# Autodesk Inventor assembly: GFRP_T2_03
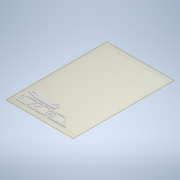
[picture p0: Inventor's stored thumbnail of the model, 180x180]
Saved by Autodesk Inventor 2020 (Build 240168000, 168)
## iProperties
Created: 2021-08-27
Part Number: GFRP_T2_03
Document SubType Name: Assembly
Designer: Masato
Author: Masato
## Documents named in this file (4)
- C:\Users\naoki\Documents\Inventor\CitBrains\git_clone\OpenPlatform4_0\CAM\OpenPlatform_ver3_0\cam\GFRP_T2_03.iam
- C:\Users\naoki\Documents\Inventor\CitBrains\git_clone\OpenPlatform4_0\ver4_0_cam_branch\OpenPlatform_ver3_0\cam\Disposable_Board.ipt
- C:\Users\naoki\Documents\Inventor\CitBrains\git_clone\OpenPlatform4_0\ver4_0_cam_branch\OpenPlatform_ver3_0\UpperBody\Arm\UpperArm_side_frame.ipt
- C:\Users\naoki\Documents\Inventor\CitBrains\git_clone\OpenPlatform4_0\ver4_0_cam_branch\OpenPlatform_ver3_0\UpperBody\Arm\ForeArm_inside_frame.ipt
## Components (5 placed, 3 different names)
1. Disposable_Board:1 — メイト:2, メイト:1, フラッシュ:1, フラッシュ:2, フラッシュ:3, フラッシュ:4
2. ForeArm_inside_frame:1 — メイト:4, フラッシュ:6, メイト:7
3. UpperArm_side_frame:2 — メイト:6, フラッシュ:5, 正接:1, メイト:9, フラッシュ:7
4. UpperArm_side_frame:1 — メイト:5, フラッシュ:3, フラッシュ:4, 正接:1, フラッシュ:5, フラッシュ:6, メイト:7
5. UpperArm_side_frame:3 — メイト:8, メイト:9, フラッシュ:7
## Relationships (16: Mate 8, Flush 7, Tangent 1)
- メイト:2 [Mate]: Disposable_Board:1
- メイト:1 [Mate]: Disposable_Board:1
- フラッシュ:1 [Flush]: Disposable_Board:1
- フラッシュ:2 [Flush]: Disposable_Board:1
- メイト:4 [Mate]: ForeArm_inside_frame:1
- メイト:5 [Mate]: UpperArm_side_frame:1
- フラッシュ:3 [Flush] (2 mm): Disposable_Board:1 ↔ UpperArm_side_frame:1
- フラッシュ:4 [Flush] (2 mm): Disposable_Board:1 ↔ UpperArm_side_frame:1
- メイト:6 [Mate]: UpperArm_side_frame:2
- フラッシュ:5 [Flush]: UpperArm_side_frame:2 ↔ UpperArm_side_frame:1
- 正接:1 [Tangent] (2.5 mm): UpperArm_side_frame:2 ↔ UpperArm_side_frame:1
- フラッシュ:6 [Flush]: ForeArm_inside_frame:1 ↔ UpperArm_side_frame:1
- メイト:7 [Mate] (2.5 mm): ForeArm_inside_frame:1 ↔ UpperArm_side_frame:1
- メイト:8 [Mate]: UpperArm_side_frame:3
- メイト:9 [Mate] (2.5 mm): UpperArm_side_frame:2 ↔ UpperArm_side_frame:3
- フラッシュ:7 [Flush]: UpperArm_side_frame:2 ↔ UpperArm_side_frame:3
